# Autodesk Inventor assembly: Złożenie gripper
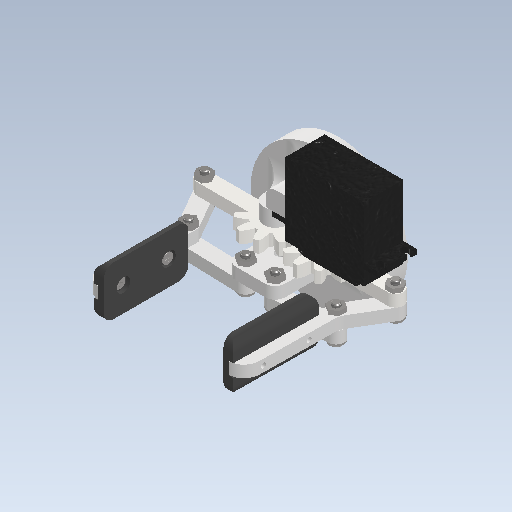
[picture p0: Inventor's stored thumbnail of the model, 512x512]
Saved by Autodesk Inventor 2021 (Build 250183000, 183)
## iProperties
Created: 2022-01-08
Part Number: Złożenie gripper
Document SubType Name: Assembly
Designer: Łukasz
Author: Łukasz
## Documents named in this file (11)
- E:\GITHUB_Czołg\Szybki-Czolg-antyRadziecki\Ramie robota\Ramie robota\Złożenie gripper.iam
- E:\GITHUB_Czołg\Szybki-Czolg-antyRadziecki\Ramie robota\Ramie robota\Gripper 5-1.ipt
- E:\GITHUB_Czołg\Szybki-Czolg-antyRadziecki\Ramie robota\Ramie robota\servo 20x40.ipt
- E:\GITHUB_Czołg\Szybki-Czolg-antyRadziecki\Ramie robota\Ramie robota\przekładnia gripper\Design Accelerator\Spur Gear15.ipt
- E:\GITHUB_Czołg\Szybki-Czolg-antyRadziecki\Ramie robota\Ramie robota\przekładnia gripper\Design Accelerator\Spur Gear25.ipt
- E:\GITHUB_Czołg\Szybki-Czolg-antyRadziecki\Ramie robota\Ramie robota\Gripper 5-2.ipt
- E:\GITHUB_Czołg\Szybki-Czolg-antyRadziecki\Ramie robota\Ramie robota\Gripper 5-3.ipt
- C:\Users\Łukasz\Documents\Inventor\Content Center Files\R2021\en-US\AS 1427(05)\AS 1427 - M4 x 16(5) II.ipt
- C:\Users\Łukasz\Documents\Inventor\Content Center Files\R2021\en-US\AS 1474(1)\AS 1474 - M4(1).ipt
- E:\GITHUB_Czołg\Szybki-Czolg-antyRadziecki\Ramie robota\Ramie robota\Gripper 5-4.ipt
- C:\Users\Łukasz\Documents\Inventor\Content Center Files\R2021\en-US\AS 1427(04)\AS 1427 - M3 x 5(5) I.ipt
## Components (27 placed, 10 different names)
1. Gripper 5-1:1 — Mate:1, Mate:2, Mate:6, Mate:7, Mate:8, Mate:16, Mate:17, Mate:19, Mate:21, Angle:1, Angle:2, Rigid:10, Rigid:11
2. servo 20x40:1 — Mate:1, Mate:2, Mate:6, Mate:9
3. Spur Gear1:1 — Mate:9, Flush:1, Mate:12, Mate:13, Angle:2, Rotation:1, Rigid:8
4. Spur Gear2:1 — Mate:7, Mate:8, Flush:1, Mate:10, Mate:14, Mate:15, Angle:1, Rotation:1, Rigid:7, Rigid:13
5. Gripper 5-2:1 — Mate:10, Mate:14, Mate:15, Mate:22, Rigid:6, Rigid:12, Rotational:1, Rotational:2
6. Gripper 5-2:2 — Mate:12, Mate:13, Mate:18, Rigid:1, Rigid:9, Rotational:3, Rotational:4
7. Gripper 5-3:1 — Mate:16, Mate:17, Mate:18, Rigid:2, Rigid:3
8. Gripper 5-3:2 — Mate:19, Mate:21, Mate:22, Rigid:4, Rigid:5
9. AS 1427 H - Metric M4 x 16:1 — Rigid:1
10. AS 1427 H - Metric M4 x 16:2 — Rigid:2
11. AS 1427 H - Metric M4 x 16:3 — Rigid:3
12. AS 1427 H - Metric M4 x 16:4 — Rigid:5
13. AS 1427 H - Metric M4 x 16:5 — Rigid:4
14. AS 1427 H - Metric M4 x 16:6 — Rigid:6
15. AS 1427 H - Metric M4 x 16:7 — Rigid:7
16. AS 1474 - Metric M4:1 — Rigid:8
17. AS 1474 - Metric M4:2 — Rigid:10
18. AS 1474 - Metric M4:3 — Rigid:9
19. AS 1474 - Metric M4:4 — Rigid:12
20. AS 1474 - Metric M4:5 — Rigid:13
21. AS 1474 - Metric M4:6 — Rigid:11
22. Gripper 5-4:1 — Rotational:3, Rotational:4, Rotational:5, Rotational:6
23. Gripper 5-4:2 — Rotational:1, Rotational:2, Rigid:14, Rotational:8
24. AS 1427 H - Metric M3 x 5:1 — Rotational:6
25. AS 1427 H - Metric M3 x 5:2 — Rotational:5
26. AS 1427 H - Metric M3 x 5:3 — Rotational:8
27. AS 1427 H - Metric M3 x 5:4 — Rigid:14
## Relationships (42: Mate 17, WeldJoint 14, RevoluteJoint 7, Angle 2, Flush 1, RelateRotation 1)
- Mate:1: Gripper 5-1:1 ↔ servo 20x40:1
- Mate:2: Gripper 5-1:1 ↔ servo 20x40:1
- Mate:6: Gripper 5-1:1 ↔ servo 20x40:1
- Mate:7: Gripper 5-1:1 ↔ Spur Gear2:1
- Mate:8: Gripper 5-1:1 ↔ Spur Gear2:1
- Mate:9: servo 20x40:1 ↔ Spur Gear1:1
- Flush:1: Spur Gear1:1 ↔ Spur Gear2:1
- Mate:10: Spur Gear2:1 ↔ Gripper 5-2:1
- Mate:12: Spur Gear1:1 ↔ Gripper 5-2:2
- Mate:13: Spur Gear1:1 ↔ Gripper 5-2:2
- Mate:14: Spur Gear2:1 ↔ Gripper 5-2:1
- Mate:15: Spur Gear2:1 ↔ Gripper 5-2:1
- Mate:16: Gripper 5-1:1 ↔ Gripper 5-3:1
- Mate:17: Gripper 5-1:1 ↔ Gripper 5-3:1
- Mate:18: Gripper 5-2:2 ↔ Gripper 5-3:1
- Mate:19: Gripper 5-1:1 ↔ Gripper 5-3:2
- Mate:21: Gripper 5-1:1 ↔ Gripper 5-3:2
- Mate:22: Gripper 5-2:1 ↔ Gripper 5-3:2
- Angle:1 (0 deg): Gripper 5-1:1 ↔ Spur Gear2:1
- Angle:2 (0 deg): Gripper 5-1:1 ↔ Spur Gear1:1
- Rotation:1 [RelateRotation] (1 ul): Spur Gear1:1 ↔ Spur Gear2:1
- Rigid:1 [WeldJoint]: Gripper 5-2:2 ↔ AS 1427 H - Metric M4 x 16:1
- Rigid:2 [WeldJoint]: Gripper 5-3:1 ↔ AS 1427 H - Metric M4 x 16:2
- Rigid:3 [WeldJoint]: Gripper 5-3:1 ↔ AS 1427 H - Metric M4 x 16:3
- Rigid:4 [WeldJoint]: Gripper 5-3:2 ↔ AS 1427 H - Metric M4 x 16:5
- Rigid:5 [WeldJoint]: Gripper 5-3:2 ↔ AS 1427 H - Metric M4 x 16:4
- Rigid:6 [WeldJoint]: Gripper 5-2:1 ↔ AS 1427 H - Metric M4 x 16:6
- Rigid:7 [WeldJoint]: Spur Gear2:1 ↔ AS 1427 H - Metric M4 x 16:7
- Rigid:8 [WeldJoint]: Spur Gear1:1 ↔ AS 1474 - Metric M4:1
- Rigid:9 [WeldJoint]: Gripper 5-2:2 ↔ AS 1474 - Metric M4:3
- Rigid:10 [WeldJoint]: Gripper 5-1:1 ↔ AS 1474 - Metric M4:2
- Rigid:11 [WeldJoint]: Gripper 5-1:1 ↔ AS 1474 - Metric M4:6
- Rigid:12 [WeldJoint]: Gripper 5-2:1 ↔ AS 1474 - Metric M4:4
- Rigid:13 [WeldJoint]: Spur Gear2:1 ↔ AS 1474 - Metric M4:5
- Rotational:1 [RevoluteJoint]: Gripper 5-2:1 ↔ Gripper 5-4:2
- Rotational:2 [RevoluteJoint]: Gripper 5-2:1 ↔ Gripper 5-4:2
- Rotational:3 [RevoluteJoint]: Gripper 5-2:2 ↔ Gripper 5-4:1
- Rotational:4 [RevoluteJoint]: Gripper 5-2:2 ↔ Gripper 5-4:1
- Rigid:14 [WeldJoint]: Gripper 5-4:2 ↔ AS 1427 H - Metric M3 x 5:4
- Rotational:5 [RevoluteJoint]: Gripper 5-4:1 ↔ AS 1427 H - Metric M3 x 5:2
- Rotational:6 [RevoluteJoint]: Gripper 5-4:1 ↔ AS 1427 H - Metric M3 x 5:1
- Rotational:8 [RevoluteJoint]: Gripper 5-4:2 ↔ AS 1427 H - Metric M3 x 5:3
